# Autodesk Inventor assembly: MountedMotor
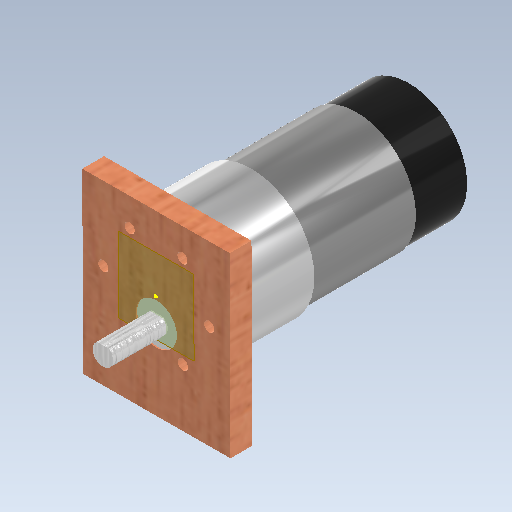
[picture p0: Inventor's stored thumbnail of the model, 512x512]
Saved by Autodesk Inventor 2021 (Build 250183000, 183)
## iProperties
Created: 2021-02-02
Part Number: MountedMotor
Document SubType Name: Assembly
Designer: garre
Author: garre
## Documents named in this file (3)
- C:\Users\Ryan\Documents\School\MQP\Case Model\Branch2\MQPInstrumentCAD-bodyModification\MQPInstrumentCAD-bodyModification\MountedMotor.iam
- C:\Users\Ryan\Documents\School\MQP\Case Model\Branch2\MQPInstrumentCAD-bodyModification\MQPInstrumentCAD-bodyModification\Motor.ipt
- C:\Users\Ryan\Documents\School\MQP\Case Model\Branch2\MQPInstrumentCAD-bodyModification\MQPInstrumentCAD-bodyModification\MotorMount.ipt
## Components (2 placed, 2 different names)
1. Motor:1 — Mate:1, Mate:2, Mate:3
2. MotorMount:1 — Mate:1, Mate:2, Mate:3
## Relationships (3: Mate 3)
- Mate:1: Motor:1 ↔ MotorMount:1
- Mate:2: Motor:1 ↔ MotorMount:1
- Mate:3: Motor:1 ↔ MotorMount:1
